# Autodesk Inventor assembly: counterweight-asm
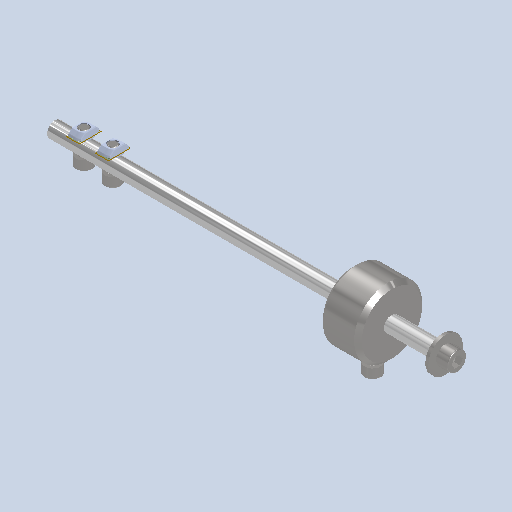
[picture p0: Inventor's stored thumbnail of the model, 512x512]
Saved by Autodesk Inventor 2024 (Build 280153000, 153)
## iProperties
Created: 2025-12-27
Part Number: counterweight-asm
Document SubType Name: Assembly
Designer: schar
Author: schar
## Documents named in this file (8)
- C:\Users\schar\Desktop\projectBlueprint\AMSTS\hardware\counterweight-asm.iam
- C:\Users\schar\Desktop\projectBlueprint\AMSTS\hardware\counterweight-rod.ipt
- C:\Users\schar\Documents\Inventor\Content Center Files\R2024\en-US\DIN 9021\DIN 9021 - 6,4.ipt
- C:\Users\schar\Documents\Inventor\Content Center Files\R2024\en-US\ISO 4762(1)\DIN EN ISO 4762 - M6 x 10.ipt
- C:\Users\schar\Desktop\projectBlueprint\AMSTS\hardware\counterweight#.ipt
- C:\Users\schar\Documents\Inventor\Content Center Files\R2024\en-US\ISO 4762(1)\DIN EN ISO 4762 - M5 x 16.ipt
- C:\Users\schar\Desktop\projectBlueprint\AMSTS\hardware\tnut_m5_2020.ipt
- C:\Users\schar\Documents\Inventor\Content Center Files\R2024\en-US\ISO 4762(1)\DIN EN ISO 4762 - M5 x 12.ipt
## Components (9 placed, 7 different names)
1. counterweight-rod:1 — Mate:1, Mate:2, Mate:3, Mate:5, Rigid:1, Rigid:2, Mate:8, Mate:9
2. DIN 9021 6,4:1 — Mate:1, Mate:2, Mate:4
3. DIN EN ISO 4762 M6 x 10:1 — Mate:3, Mate:4
4. counterweight#:1 — Mate:5, Mate:6, Mate:7
5. DIN EN ISO 4762 M5 x 16:1 — Mate:6, Mate:7
6. tnut_m5_2020:1 — Rigid:1, Flush:1
7. tnut_m5_2020:2 — Rigid:2, Flush:2
8. DIN EN ISO 4762 M5 x 12:1 — Mate:8, Flush:1
9. DIN EN ISO 4762 M5 x 12:2 — Mate:9, Flush:2
## Relationships (13: Mate 9, WeldJoint 2, Flush 2)
- Mate:1: counterweight-rod:1 ↔ DIN 9021 6,4:1
- Mate:2: counterweight-rod:1 ↔ DIN 9021 6,4:1
- Mate:3: counterweight-rod:1 ↔ DIN EN ISO 4762 M6 x 10:1
- Mate:4: DIN 9021 6,4:1 ↔ DIN EN ISO 4762 M6 x 10:1
- Mate:5: counterweight-rod:1 ↔ counterweight#:1
- Mate:6: counterweight#:1 ↔ DIN EN ISO 4762 M5 x 16:1
- Mate:7 (22 mm): counterweight#:1 ↔ DIN EN ISO 4762 M5 x 16:1
- Rigid:1 [WeldJoint]: counterweight-rod:1 ↔ tnut_m5_2020:1
- Rigid:2 [WeldJoint]: counterweight-rod:1 ↔ tnut_m5_2020:2
- Mate:8: counterweight-rod:1 ↔ DIN EN ISO 4762 M5 x 12:1
- Flush:1: tnut_m5_2020:1 ↔ DIN EN ISO 4762 M5 x 12:1
- Mate:9: counterweight-rod:1 ↔ DIN EN ISO 4762 M5 x 12:2
- Flush:2: tnut_m5_2020:2 ↔ DIN EN ISO 4762 M5 x 12:2
